# Autodesk Inventor assembly: avionics_reassemb
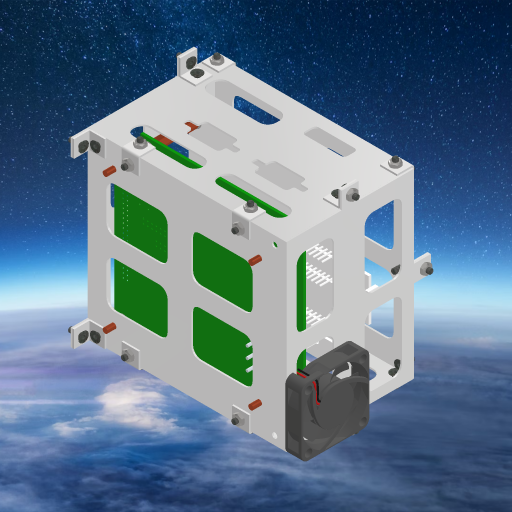
[picture p0: Inventor's stored thumbnail of the model, 512x512]
Saved by Autodesk Inventor 2023 (Build 270158000, 158)
## iProperties
Created: 2023-10-19
Part Number: avionics_reassemb
Document SubType Name: Assembly
Designer: 310611102
Mass: 284.721 g
Surface Area: 1403.32 cm^2
Volume: 70.7972 cm^3
Density: 4.02164 g/cm^3
Author: 310611102
## Documents named in this file (12)
- C:\Users\310611102\Documents\Inventor\SSR\avionics_2023ver\assembly\avionics_reassemb.iam
- C:\Users\310611102\Documents\Inventor\SSR\avionics_2023ver\electronics\shield box\shieldbox_ver2\PCB_board_box_reassemb.iam
- C:\Users\310611102\Documents\Inventor\SSR\avionics_2023ver\electronics\Power_supply_board.ipt
- C:\Users\310611102\Documents\Inventor\SSR\avionics_2023ver\electronics\copper_pillar_M3_L4.ipt
- C:\Users\310611102\Documents\Inventor\SSR\avionics_2023ver\electronics\washerM3x0.5h.ipt
- C:\Users\310611102\Documents\Inventor\SSR\avionics_2023ver\electronics\copper_pillar_M3_L15.ipt
- C:\Users\310611102\Documents\Inventor\SSR\avionics_2023ver\electronics\STM32 Communication Board ver1.0.ipt
- C:\Users\310611102\Documents\Inventor\SSR\avionics_2023ver\electronics\copper_pillar_M3_L25.ipt
- C:\Users\310611102\Documents\Inventor\SSR\avionics_2023ver\electronics\empty_board.ipt
- C:\Users\310611102\Documents\Inventor\SSR\avionics_2023ver\electronics\MTI-7\MTi 1-series v3.iam
- C:\Users\310611102\Documents\Inventor\SSR\avionics_2023ver\electronics\ISO 4032 - M3 - ISO.ipt
- C:\Users\310611102\Documents\Inventor\SSR\avionics_2023ver\electronics\cooling_fan.ipt
## Components (42 placed, 11 different names)
1. PCB_board_box_reassemb:1 [sub-assembly] — Insert:1, Insert:2, Insert:3, Insert:4, Insert:48, Insert:49
2. Power_supply_board:1 — Insert:9, Insert:10, Insert:14, Insert:16, Insert:18, Insert:20
3. copper_pillar_M3_L4:1 — Insert:1, Insert:6
4. copper_pillar_M3_L4:2 — Insert:3, Insert:7
5. copper_pillar_M3_L4:3 — Insert:4, Insert:8
6. copper_pillar_M3_L4:4 — Insert:2, Insert:5
7. washerM3x0.5h:1 — Insert:5
8. washerM3x0.5h:2 — Insert:6, Insert:9
9. washerM3x0.5h:3 — Insert:7
10. washerM3x0.5h:4 — Insert:8, Insert:10
11. copper_pillar_M3_L15:1 — Insert:19, Insert:24
12. copper_pillar_M3_L15:2 — Insert:21, Insert:25
13. copper_pillar_M3_L15:3 — Insert:15, Insert:22
14. copper_pillar_M3_L15:4 — Insert:17, Insert:23
15. washerM3x0.5h:5 — Insert:14, Insert:15
16. washerM3x0.5h:6 — Insert:16, Insert:17
17. washerM3x0.5h:7 — Insert:18, Insert:19
18. washerM3x0.5h:8 — Insert:20, Insert:21
19. washerM3x0.5h:9 — Insert:22
20. washerM3x0.5h:10 — Insert:23, Insert:27
21. washerM3x0.5h:11 — Insert:24, Insert:26
22. washerM3x0.5h:12 — Insert:25
23. STM32 Communication Board ver1.0:1 — Insert:26, Insert:27, Insert:28, Insert:29, Insert:30, Insert:31
24. washerM3x0.5h:13 — Insert:28, Insert:33
25. washerM3x0.5h:14 — Insert:29, Insert:32
26. washerM3x0.5h:15 — Insert:30, Insert:34
27. washerM3x0.5h:16 — Insert:31, Insert:35
28. copper_pillar_M3_L25:1 — Insert:32, Insert:39
29. copper_pillar_M3_L25:2 — Insert:33, Insert:37
30. copper_pillar_M3_L25:3 — Insert:34, Insert:36
31. copper_pillar_M3_L25:4 — Insert:35, Insert:38
32. washerM3x0.5h:17 — Insert:36
33. washerM3x0.5h:18 — Insert:38
34. washerM3x0.5h:19 — Insert:37, Insert:40
35. washerM3x0.5h:20 — Insert:39, Insert:41
36. empty_board:1 — Insert:40, Insert:41, Insert:42, Insert:43, Insert:44, Insert:45, Insert:46
37. MTi 1-series v3:1 [sub-assembly] — Insert:42, Insert:43, Insert:47
38. ISO 4032 M3:1 — Insert:44
39. ISO 4032 M3:2 — Insert:45
40. ISO 4032 M3:3 — Insert:47
41. ISO 4032 M3:4 — Insert:46
42. cooling_fan:1 — Insert:48, Insert:49
## Relationships (46: Insert 46)
- Insert:1: PCB_board_box_reassemb:1 ↔ copper_pillar_M3_L4:1
- Insert:2: PCB_board_box_reassemb:1 ↔ copper_pillar_M3_L4:4
- Insert:3: PCB_board_box_reassemb:1 ↔ copper_pillar_M3_L4:2
- Insert:4: PCB_board_box_reassemb:1 ↔ copper_pillar_M3_L4:3
- Insert:5: copper_pillar_M3_L4:4 ↔ washerM3x0.5h:1
- Insert:6: copper_pillar_M3_L4:1 ↔ washerM3x0.5h:2
- Insert:7: copper_pillar_M3_L4:2 ↔ washerM3x0.5h:3
- Insert:8: copper_pillar_M3_L4:3 ↔ washerM3x0.5h:4
- Insert:9: Power_supply_board:1 ↔ washerM3x0.5h:2
- Insert:10: Power_supply_board:1 ↔ washerM3x0.5h:4
- Insert:14: Power_supply_board:1 ↔ washerM3x0.5h:5
- Insert:15: copper_pillar_M3_L15:3 ↔ washerM3x0.5h:5
- Insert:16: Power_supply_board:1 ↔ washerM3x0.5h:6
- Insert:17: copper_pillar_M3_L15:4 ↔ washerM3x0.5h:6
- Insert:18: Power_supply_board:1 ↔ washerM3x0.5h:7
- Insert:19: copper_pillar_M3_L15:1 ↔ washerM3x0.5h:7
- Insert:20: Power_supply_board:1 ↔ washerM3x0.5h:8
- Insert:21: copper_pillar_M3_L15:2 ↔ washerM3x0.5h:8
- Insert:22: copper_pillar_M3_L15:3 ↔ washerM3x0.5h:9
- Insert:23: copper_pillar_M3_L15:4 ↔ washerM3x0.5h:10
- Insert:24: copper_pillar_M3_L15:1 ↔ washerM3x0.5h:11
- Insert:25: copper_pillar_M3_L15:2 ↔ washerM3x0.5h:12
- Insert:26: washerM3x0.5h:11 ↔ STM32 Communication Board ver1.0:1
- Insert:27: washerM3x0.5h:10 ↔ STM32 Communication Board ver1.0:1
- Insert:28: STM32 Communication Board ver1.0:1 ↔ washerM3x0.5h:13
- Insert:29: STM32 Communication Board ver1.0:1 ↔ washerM3x0.5h:14
- Insert:30: STM32 Communication Board ver1.0:1 ↔ washerM3x0.5h:15
- Insert:31: STM32 Communication Board ver1.0:1 ↔ washerM3x0.5h:16
- Insert:32: washerM3x0.5h:14 ↔ copper_pillar_M3_L25:1
- Insert:33: washerM3x0.5h:13 ↔ copper_pillar_M3_L25:2
- Insert:34: washerM3x0.5h:15 ↔ copper_pillar_M3_L25:3
- Insert:35: washerM3x0.5h:16 ↔ copper_pillar_M3_L25:4
- Insert:36: copper_pillar_M3_L25:3 ↔ washerM3x0.5h:17
- Insert:37: copper_pillar_M3_L25:2 ↔ washerM3x0.5h:19
- Insert:38: copper_pillar_M3_L25:4 ↔ washerM3x0.5h:18
- Insert:39: copper_pillar_M3_L25:1 ↔ washerM3x0.5h:20
- Insert:40: washerM3x0.5h:19 ↔ empty_board:1
- Insert:41: washerM3x0.5h:20 ↔ empty_board:1
- Insert:42: empty_board:1 ↔ MTi 1-series v3:1
- Insert:43: empty_board:1 ↔ MTi 1-series v3:1
- Insert:44: empty_board:1 ↔ ISO 4032 M3:1
- Insert:45: empty_board:1 ↔ ISO 4032 M3:2
- Insert:46: empty_board:1 ↔ ISO 4032 M3:4
- Insert:47: MTi 1-series v3:1 ↔ ISO 4032 M3:3
- Insert:48: PCB_board_box_reassemb:1 ↔ cooling_fan:1
- Insert:49: PCB_board_box_reassemb:1 ↔ cooling_fan:1
